# Autodesk Inventor assembly: Assembly2
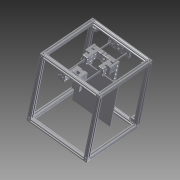
[picture p0: Inventor's stored thumbnail of the model, 180x180]
Saved by Autodesk Inventor 2012 (Build 160160000, 160)
## iProperties
Created: 2013-02-04
Part Number: Assembly2
Document SubType Name: Assembly
Designer: mce
Mass: 1579.2 g
Surface Area: 10222.6 cm^2
Volume: 1579.2 cm^3
Density: 1 g/cm^3
Author: mce
## Documents named in this file (28)
- D:\Perso 3D\Printer Home\Zaxe\Assembly2.iam
- D:\Perso 3D\Printer Home\Zaxe\Z move clamp small.ipt
- D:\Perso 3D\Printer Home\Zaxe\Z move left.ipt
- D:\Perso 3D\Printer Home\Zaxe\Z move clamp.ipt
- D:\Perso 3D\Printer Home\Zaxe\Z move middle.ipt
- D:\Perso 3D\Printer Home\Zaxe\V5 Z Top.ipt
- D:\Perso 3D\Printer Home\Zaxe\lm8uu.ipt
- D:\Perso 3D\Printer Home\Zaxe\V5 Z Bottom.ipt
- D:\Perso 3D\Printer Home\Zaxe\V5 Z Spacer.ipt
- D:\Perso 3D\Printer Home\Zaxe\V5 Z Bottom Center.ipt
- D:\Perso 3D\Printer Home\Zaxe\Plate.ipt
- D:\Perso 3D\Printer Home\Zaxe\V5 Z Top bearing.ipt
- D:\Perso 3D\Printer Home\Zaxe\Z move plate.ipt
- D:\Perso 3D\Printer Home\Zaxe\Set Square.ipt
- D:\Perso 3D\profile.ipt
- D:\Perso 3D\Corner Profile.ipt
- D:\Perso 3D\profile350mm.ipt
- D:\Perso 3D\Printer Home\Zaxe\Rod.ipt
- D:\Perso 3D\PiedClip.ipt
- D:\Perso 3D\Silenbloc.ipt
- D:\Perso 3D\Printer Home\Zaxe\Assembly2\AIP\FEA\ant0a64gw.fins
- D:\Perso 3D\Printer Home\Zaxe\Assembly2\AIP\FEA\ant0a64gw.fsat
- D:\Perso 3D\Printer Home\Zaxe\Assembly2\AIP\FEA\ant0a64gw.ftes
- D:\Perso 3D\Printer Home\Zaxe\Assembly2\AIP\FEA\ant0a64gw.fwiz
- D:\Perso 3D\Printer Home\Zaxe\Assembly2\AIP\FEA\ant0a654w.fmsh
- D:\Perso 3D\Printer Home\Zaxe\Assembly2\AIP\FEA\ant0a654x.fres
- D:\Perso 3D\Printer Home\Zaxe\Assembly2\AIP\FEA\ant0a660w.fmsh
- D:\Perso 3D\Printer Home\Zaxe\Assembly2\AIP\FEA\ant0a660x.fres
## Components (57 placed, 19 different names)
1. Z move clamp small:1 — Flush:1, Mate:2, Flush:1
2. Z move left:1 — Flush:1, Mate:2, Flush:1, Flush:6, Flush:7, Mate:7, Flush:9, Mate:8, Mate:28, Flush:35, Flush:39, Mate:31, Mate:32, Flush:41, Flush:44, Flush:46
3. Z move middle:1 — Flush:6, Flush:8, Mate:27, Mate:28, Flush:34, Flush:35, Mate:42, Mate:97
4. Z move left:2 — Flush:8, Flush:10, Mate:9, Mate:10, Flush:11, Flush:12, Flush:13, Mate:11, Mate:27, Flush:34, Flush:40, Mate:33, Mate:34, Flush:42, Flush:43, Flush:45
5. V5 Z Top:1 — Mate:24, Flush:29, Flush:30, Flush:37, Mate:30, Flush:38
6. lm8uu:1 — Flush:7, Mate:7, Mate:75
7. lm8uu:2 — Flush:9, Mate:8, Mate:77
8. lm8uu:3 — Mate:10, Flush:11, Mate:74
9. lm8uu:4 — Flush:10, Mate:9, Mate:76
10. Z move clamp small:2 — Flush:12, Flush:13, Mate:11
11. V5 Z Bottom:1 — Mate:15, Flush:18, Mate:18, Flush:21, Flush:24, Flush:25, Mate:21, Flush:27, Mate:25, Mate:67
12. V5 Z Bottom:2 — Mate:12, Flush:17, Mate:19, Flush:22, Flush:24, Mate:21, Flush:27, Flush:31, Flush:32
13. V5 Z Bottom:3 — Mate:13, Flush:20, Mate:19, Flush:22, Flush:26, Mate:24, Flush:29, Mate:50
14. V5 Z Bottom:4 — Mate:14, Flush:19, Mate:18, Flush:21, Flush:25, Flush:26, Flush:30
15. V5 Z Spacer:1 — Mate:15, Flush:18, Mate:71, Mate:73
16. V5 Z Spacer:2 — Mate:14, Flush:19, Mate:70
17. V5 Z Spacer:3 — Mate:13, Flush:20, Mate:69, Mate:72
18. V5 Z Spacer:4 — Mate:12, Flush:17, Mate:68
19. V5 Z Bottom Center:1 — Mate:25, Flush:31, Flush:32, Flush:63, Mate:97
20. Plate:1 — Mate:41, Mate:42, Flush:47
21. V5 Z Top bearing:1 — Flush:37, Mate:30, Flush:38
22. Z move clamp:3 — Flush:39, Mate:31, Mate:32, Mate:35, Mate:36, Mate:37
23. Z move clamp:5 — Flush:40, Mate:33, Mate:34, Mate:38, Mate:39, Mate:40
24. Z move plate:1 — Flush:41, Flush:44, Flush:46
25. Z move plate:2 — Flush:42, Flush:43, Flush:45
26. Set Square:1 — Mate:35, Mate:36, Mate:37, Mate:41, Flush:47
27. Set Square:2 — Mate:38, Mate:39, Mate:40
28. profile:1 — Mate:46, Flush:47, Flush:54, Mate:47, Flush:55, Flush:56
29. profile:2 — Mate:49, Flush:59, Flush:60, Flush:61, Flush:62, Flush:63
30. profile:3 — Mate:63, Mate:64, Flush:88, Flush:89, Flush:90, Flush:91
31. profile:4 — Mate:61, Mate:62, Flush:84, Flush:85, Flush:86, Flush:87
32. profile:5 — Mate:43, Flush:48, Flush:49, Mate:48, Flush:57, Flush:58
33. profile:6 — Mate:59, Mate:60, Flush:80, Flush:81, Flush:82, Flush:83
34. profile:7 — Mate:44, Flush:50, Flush:51, Mate:45, Flush:52, Flush:53, Mate:50
35. profile:8 — Mate:65, Mate:66, Flush:92, Flush:93, Flush:94, Flush:95
36. Corner Profile:1 — Mate:47, Flush:55, Flush:56, Mate:49, Flush:59, Flush:60, Mate:53, Flush:68, Flush:69
37. Corner Profile:2 — Mate:45, Flush:52, Flush:53, Mate:46, Flush:47, Flush:54, Mate:51, Flush:64, Flush:65
38. Corner Profile:3 — Mate:56, Flush:74, Flush:75, Mate:61, Flush:84, Flush:85, Mate:66, Flush:92, Flush:93
39. Corner Profile:4 — Mate:57, Flush:76, Flush:77, Mate:59, Flush:80, Flush:81, Mate:63, Flush:90, Flush:91
40. Corner Profile:5 — Mate:43, Flush:48, Flush:49, Mate:44, Flush:50, Flush:51, Mate:52, Flush:66, Flush:67
41. Corner Profile:6 — Mate:48, Flush:57, Flush:58, Flush:61, Flush:62, Mate:54, Flush:70, Flush:71, Mate:88
42. Corner Profile:7 — Mate:58, Flush:78, Flush:79, Mate:62, Flush:86, Flush:87, Mate:64, Flush:88, Flush:89
43. Corner Profile:8 — Mate:55, Flush:72, Flush:73, Mate:60, Flush:82, Flush:83, Mate:65, Flush:94, Flush:95
44. profile350mm:1 — Mate:51, Flush:64, Flush:65, Mate:57, Flush:76, Flush:77
45. profile350mm:2 — Mate:52, Flush:66, Flush:67, Mate:55, Flush:72, Flush:73
46. profile350mm:3 — Mate:53, Flush:68, Flush:69, Mate:58, Flush:78, Flush:79, Mate:93, Mate:94, Mate:95, Mate:96
47. profile350mm:4 — Mate:54, Flush:70, Flush:71, Mate:56, Flush:74, Flush:75, Mate:67, Mate:82, Mate:83, Mate:86, Mate:87
48. Rod:1 — Mate:70, Mate:71, Mate:73, Mate:74, Mate:76
49. Rod:2 — Mate:68, Mate:69, Mate:72, Mate:75, Mate:77
50. PiedClip:1 — Mate:80, Mate:81, Mate:82, Mate:83, Mate:88
51. Silenbloc:1 — Mate:80, Mate:81
52. PiedClip:2 — Mate:84, Mate:85, Mate:86, Mate:87
53. Silenbloc:2 — Mate:84, Mate:85
54. PiedClip:3 — Mate:89, Mate:90, Mate:95, Mate:96
55. Silenbloc:3 — Mate:89, Mate:90
56. PiedClip:4 — Mate:91, Mate:92, Mate:93, Mate:94
57. Silenbloc:4 — Mate:91, Mate:92
## Relationships (169: Flush 86, Mate 83)
- Flush:1: Z move clamp small:1 ↔ Z move left:1
- Mate:2 (0.5 mm): Z move clamp small:1 ↔ Z move left:1
- Flush:1: Z move clamp small:1 ↔ Z move left:1
- Flush:6: Z move left:1 ↔ Z move middle:1
- Flush:8: Z move middle:1 ↔ Z move left:2
- Flush:7: Z move left:1 ↔ lm8uu:1
- Mate:7: Z move left:1 ↔ lm8uu:1
- Flush:9: Z move left:1 ↔ lm8uu:2
- Mate:8: Z move left:1 ↔ lm8uu:2
- Flush:10: Z move left:2 ↔ lm8uu:4
- Mate:9: Z move left:2 ↔ lm8uu:4
- Mate:10: Z move left:2 ↔ lm8uu:3
- Flush:11: Z move left:2 ↔ lm8uu:3
- Flush:12: Z move left:2 ↔ Z move clamp small:2
- Flush:13: Z move left:2 ↔ Z move clamp small:2
- Mate:11 (0.5 mm): Z move left:2 ↔ Z move clamp small:2
- Mate:12: V5 Z Bottom:2 ↔ V5 Z Spacer:4
- Mate:13: V5 Z Bottom:3 ↔ V5 Z Spacer:3
- Mate:14: V5 Z Bottom:4 ↔ V5 Z Spacer:2
- Mate:15: V5 Z Bottom:1 ↔ V5 Z Spacer:1
- Flush:17: V5 Z Bottom:2 ↔ V5 Z Spacer:4
- Flush:18: V5 Z Bottom:1 ↔ V5 Z Spacer:1
- Flush:19: V5 Z Bottom:4 ↔ V5 Z Spacer:2
- Flush:20: V5 Z Bottom:3 ↔ V5 Z Spacer:3
- Mate:18 (300 mm): V5 Z Bottom:1 ↔ V5 Z Bottom:4
- Mate:19 (300 mm): V5 Z Bottom:2 ↔ V5 Z Bottom:3
- Flush:21: V5 Z Bottom:1 ↔ V5 Z Bottom:4
- Flush:22: V5 Z Bottom:2 ↔ V5 Z Bottom:3
- Flush:24: V5 Z Bottom:1 ↔ V5 Z Bottom:2
- Flush:25: V5 Z Bottom:1 ↔ V5 Z Bottom:4
- Mate:21 (60 mm): V5 Z Bottom:1 ↔ V5 Z Bottom:2
- Flush:26: V5 Z Bottom:3 ↔ V5 Z Bottom:4
- Flush:27: V5 Z Bottom:1 ↔ V5 Z Bottom:2
- Mate:24: V5 Z Top:1 ↔ V5 Z Bottom:3
- Flush:29: V5 Z Top:1 ↔ V5 Z Bottom:3
- Flush:30: V5 Z Top:1 ↔ V5 Z Bottom:4
- Mate:25: V5 Z Bottom:1 ↔ V5 Z Bottom Center:1
- Flush:31: V5 Z Bottom:2 ↔ V5 Z Bottom Center:1
- Flush:32: V5 Z Bottom:2 ↔ V5 Z Bottom Center:1
- Mate:27: Z move middle:1 ↔ Z move left:2
- Mate:28: Z move left:1 ↔ Z move middle:1
- Flush:34: Z move middle:1 ↔ Z move left:2
- Flush:35: Z move left:1 ↔ Z move middle:1
- Flush:37: V5 Z Top:1 ↔ V5 Z Top bearing:1
- Mate:30: V5 Z Top:1 ↔ V5 Z Top bearing:1
- Flush:38: V5 Z Top:1 ↔ V5 Z Top bearing:1
- Flush:39: Z move left:1 ↔ Z move clamp:3
- Mate:31: Z move left:1 ↔ Z move clamp:3
- Mate:32: Z move left:1 ↔ Z move clamp:3
- Flush:40: Z move left:2 ↔ Z move clamp:5
- Mate:33: Z move left:2 ↔ Z move clamp:5
- Mate:34: Z move left:2 ↔ Z move clamp:5
- Flush:41: Z move left:1 ↔ Z move plate:1
- Flush:42: Z move left:2 ↔ Z move plate:2
- Flush:43: Z move left:2 ↔ Z move plate:2
- Flush:44: Z move left:1 ↔ Z move plate:1
- Flush:45: Z move left:2 ↔ Z move plate:2
- Flush:46: Z move left:1 ↔ Z move plate:1
- Mate:35: Z move clamp:3 ↔ Set Square:1
- Mate:36: Z move clamp:3 ↔ Set Square:1
- Mate:37: Z move clamp:3 ↔ Set Square:1
- Mate:38: Z move clamp:5 ↔ Set Square:2
- Mate:39: Z move clamp:5 ↔ Set Square:2
- Mate:40: Z move clamp:5 ↔ Set Square:2
- Mate:41: Plate:1 ↔ Set Square:1
- Mate:42 (-340 mm): Z move middle:1 ↔ Plate:1
- Flush:47 (37.5 mm): Plate:1 ↔ Set Square:1
- Mate:43: profile:5 ↔ Corner Profile:5
- Flush:48: profile:5 ↔ Corner Profile:5
- Flush:49: profile:5 ↔ Corner Profile:5
- Mate:44: profile:7 ↔ Corner Profile:5
- Flush:50: profile:7 ↔ Corner Profile:5
- Flush:51: profile:7 ↔ Corner Profile:5
- Mate:45: profile:7 ↔ Corner Profile:2
- Flush:52: profile:7 ↔ Corner Profile:2
- Flush:53: profile:7 ↔ Corner Profile:2
- Mate:46: profile:1 ↔ Corner Profile:2
- Flush:47: profile:1 ↔ Corner Profile:2
- Flush:54: profile:1 ↔ Corner Profile:2
- Mate:47: profile:1 ↔ Corner Profile:1
- Flush:55: profile:1 ↔ Corner Profile:1
- Flush:56: profile:1 ↔ Corner Profile:1
- Mate:48: profile:5 ↔ Corner Profile:6
- Flush:57: profile:5 ↔ Corner Profile:6
- Flush:58: profile:5 ↔ Corner Profile:6
- Mate:49: profile:2 ↔ Corner Profile:1
- Flush:59: profile:2 ↔ Corner Profile:1
- Flush:60: profile:2 ↔ Corner Profile:1
- Flush:61: profile:2 ↔ Corner Profile:6
- Flush:62: profile:2 ↔ Corner Profile:6
- Mate:50: V5 Z Bottom:3 ↔ profile:7
- Flush:63: V5 Z Bottom Center:1 ↔ profile:2
- Mate:51: Corner Profile:2 ↔ profile350mm:1
- Flush:64: Corner Profile:2 ↔ profile350mm:1
- Flush:65: Corner Profile:2 ↔ profile350mm:1
- Mate:52: Corner Profile:5 ↔ profile350mm:2
- Flush:66: Corner Profile:5 ↔ profile350mm:2
- Flush:67: Corner Profile:5 ↔ profile350mm:2
- Mate:53: Corner Profile:1 ↔ profile350mm:3
- Flush:68: Corner Profile:1 ↔ profile350mm:3
- Flush:69: Corner Profile:1 ↔ profile350mm:3
- Mate:54: Corner Profile:6 ↔ profile350mm:4
- Flush:70: Corner Profile:6 ↔ profile350mm:4
- Flush:71: Corner Profile:6 ↔ profile350mm:4
- Mate:55: Corner Profile:8 ↔ profile350mm:2
- Flush:72: Corner Profile:8 ↔ profile350mm:2
- Flush:73: Corner Profile:8 ↔ profile350mm:2
- Mate:56: Corner Profile:3 ↔ profile350mm:4
- Flush:74: Corner Profile:3 ↔ profile350mm:4
- Flush:75: Corner Profile:3 ↔ profile350mm:4
- Mate:57: Corner Profile:4 ↔ profile350mm:1
- Flush:76: Corner Profile:4 ↔ profile350mm:1
- Flush:77: Corner Profile:4 ↔ profile350mm:1
- Mate:58: Corner Profile:7 ↔ profile350mm:3
- Flush:78: Corner Profile:7 ↔ profile350mm:3
- Flush:79: Corner Profile:7 ↔ profile350mm:3
- Mate:59: profile:6 ↔ Corner Profile:4
- Mate:60: profile:6 ↔ Corner Profile:8
- Flush:80: profile:6 ↔ Corner Profile:4
- Flush:81: profile:6 ↔ Corner Profile:4
- Flush:82: profile:6 ↔ Corner Profile:8
- Flush:83: profile:6 ↔ Corner Profile:8
- Mate:61: profile:4 ↔ Corner Profile:3
- Mate:62: profile:4 ↔ Corner Profile:7
- Flush:84: profile:4 ↔ Corner Profile:3
- Flush:85: profile:4 ↔ Corner Profile:3
- Flush:86: profile:4 ↔ Corner Profile:7
- Flush:87: profile:4 ↔ Corner Profile:7
- Mate:63: profile:3 ↔ Corner Profile:4
- Mate:64: profile:3 ↔ Corner Profile:7
- Flush:88: profile:3 ↔ Corner Profile:7
- Flush:89: profile:3 ↔ Corner Profile:7
- Flush:90: profile:3 ↔ Corner Profile:4
- Flush:91: profile:3 ↔ Corner Profile:4
- Mate:65: profile:8 ↔ Corner Profile:8
- Mate:66: profile:8 ↔ Corner Profile:3
- Flush:92: profile:8 ↔ Corner Profile:3
- Flush:93: profile:8 ↔ Corner Profile:3
- Flush:94: profile:8 ↔ Corner Profile:8
- Flush:95: profile:8 ↔ Corner Profile:8
- Mate:67 (90 mm): V5 Z Bottom:1 ↔ profile350mm:4
- Mate:68: V5 Z Spacer:4 ↔ Rod:2
- Mate:69: V5 Z Spacer:3 ↔ Rod:2
- Mate:70: V5 Z Spacer:2 ↔ Rod:1
- Mate:71: V5 Z Spacer:1 ↔ Rod:1
- Mate:72: V5 Z Spacer:3 ↔ Rod:2
- Mate:73: V5 Z Spacer:1 ↔ Rod:1
- Mate:74: lm8uu:3 ↔ Rod:1
- Mate:75: lm8uu:1 ↔ Rod:2
- Mate:76: lm8uu:4 ↔ Rod:1
- Mate:77: lm8uu:2 ↔ Rod:2
- Mate:80 (1 mm): PiedClip:1 ↔ Silenbloc:1
- Mate:81: PiedClip:1 ↔ Silenbloc:1
- Mate:82: profile350mm:4 ↔ PiedClip:1
- Mate:83: profile350mm:4 ↔ PiedClip:1
- Mate:84 (1 mm): PiedClip:2 ↔ Silenbloc:2
- Mate:85: PiedClip:2 ↔ Silenbloc:2
- Mate:86: profile350mm:4 ↔ PiedClip:2
- Mate:87: profile350mm:4 ↔ PiedClip:2
- Mate:88 (10 mm): Corner Profile:6 ↔ PiedClip:1
- Mate:89 (1 mm): PiedClip:3 ↔ Silenbloc:3
- Mate:90: PiedClip:3 ↔ Silenbloc:3
- Mate:91 (1 mm): PiedClip:4 ↔ Silenbloc:4
- Mate:92: PiedClip:4 ↔ Silenbloc:4
- Mate:93: profile350mm:3 ↔ PiedClip:4
- Mate:94: profile350mm:3 ↔ PiedClip:4
- Mate:95: profile350mm:3 ↔ PiedClip:3
- Mate:96: profile350mm:3 ↔ PiedClip:3
- Mate:97 (100 mm): Z move middle:1 ↔ V5 Z Bottom Center:1
## Named parameters: sa_0 = -723.092, sa_1 = 140.991, sa_2 = -676.21, sa_3 = -584.821, sa_4 = 58.5459, sa_5 = -7978.38, sa_6 = -977.48, sa_7 = 197.964, sa_8 = 73.1026
note: some values were not read from the file. Shown as the stored number, unit unknown: "sa_0", "sa_1", "sa_2", "sa_3", "sa_4", "sa_5", "sa_6", "sa_7", "sa_8".
